# Autodesk Inventor assembly: Deltabot - Small Model ver12
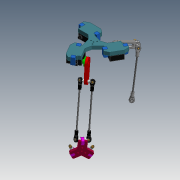
[picture p0: Inventor's stored thumbnail of the model, 180x180]
Saved by Autodesk Inventor 2014 SP1 (Build 180222100, 222)
## iProperties
Created: 2013-12-25
Part Number: Deltabot - Small Model ver12
Document SubType Name: Assembly
Designer: tom
Title: D:\My Documents\Work\GitHub\Delta_Robots\Delatabot - Small Model\Deltabot - Small Model.stp
Creation Date: 2013-12-24
Sending System: ACIS
Author: tom
## Documents named in this file (7)
- C:\Users\tom\Documents\GitHub\Delta_Robots\Delatabot - Small Model\Inventor\Deltabot - Small Model ver12\Deltabot - Small Model ver12.iam
- C:\Users\tom\Documents\GitHub\Vacubot\Inventor\Part2.ipt
- C:\Users\tom\Documents\GitHub\Delta_Robots\Delatabot - Small Model\Inventor\Deltabot - Small Model ver12\Servo_Mount.ipt
- C:\Users\tom\Documents\GitHub\Delta_Robots\Delatabot - Small Model\Inventor\Deltabot - Small Model ver12\Servo.ipt
- C:\Users\tom\Documents\GitHub\Delta_Robots\Delatabot - Small Model\Inventor\Deltabot - Small Model ver12\Servo Arm.iam
- C:\Users\tom\Documents\GitHub\Delta_Robots\Delatabot - Small Model\Inventor\Deltabot - Small Model ver12\Arm Linkage.iam
- C:\Users\tom\Documents\GitHub\Delta_Robots\Delatabot - Small Model\Inventor\Deltabot - Small Model ver12\Lower Platform Assembly.iam
## Components (16 placed, 6 different names)
1. Upper Support — Mate:15, Mate:16, Mate:17, Mate:19
2. Servo Arm:1 [sub-assembly] — Ball:1, Ball:3
3. Arm Linkage:1 [sub-assembly] — Ball:1, Ball:2
4. Lower Platform Assembly:1 [sub-assembly] — Ball:2, Ball:4
5. Arm Linkage:2 [sub-assembly] — Ball:3, Ball:4
6. Servo Arm:2 [sub-assembly] — Rotational:2, Ball:5
7. Arm Linkage:3 [sub-assembly] — Ball:5
8. Servo_Mount:1 — Mate:16, Mate:17, Mate:18, Mate:20
9. Servo_Mount:2 — Mate:15, Mate:19, Mate:21
10. Servo:1 — Mate:18, Mate:20, Mate:21
11. Servo_Mount:3
12. Servo_Mount:4
13. Servo:2
14. Servo_Mount:5
15. Servo_Mount:6
16. Servo:3 — Rotational:2
## Component patterns: (3 elements, first: Servo_Mount:1 + Servo_Mount:2 + Servo:1)
## Relationships (14: Mate 7, BallJoint 5, RevoluteJoint 2)
- Mate:15: Upper Support ↔ Servo_Mount:2
- Mate:16: Upper Support ↔ Servo_Mount:1
- Mate:17: Upper Support ↔ Servo_Mount:1
- Mate:18: Servo_Mount:1 ↔ Servo:1
- Mate:19: Upper Support ↔ Servo_Mount:2
- Mate:20: Servo_Mount:1 ↔ Servo:1
- Mate:21 (0.005 mm): Servo_Mount:2 ↔ Servo:1
- [RevoluteJoint]: Servo Arm:1 ↔ Servo:1
- Ball:1: Servo Arm:1 ↔ Arm Linkage:1
- Ball:2: Arm Linkage:1 ↔ Lower Platform Assembly:1
- Ball:3: Servo Arm:1 ↔ Arm Linkage:2
- Ball:4: Lower Platform Assembly:1 ↔ Arm Linkage:2
- Rotational:2 [RevoluteJoint]: Servo Arm:2 ↔ Servo:3
- Ball:5: Servo Arm:2 ↔ Arm Linkage:3
